# Autodesk Inventor assembly: Cube
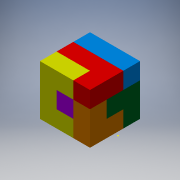
[picture p0: Inventor's stored thumbnail of the model, 180x180]
Saved by Autodesk Inventor 2017 (Build 210142000, 142)
## iProperties
Created: 2016-11-02
Part Number: Cube
Document SubType Name: Assembly
Designer: rbibb
Author: rbibb
## Documents named in this file (7)
- A:\rbibb\School\9th\Enginering\Cube.iam
- A:\rbibb\School\9th\Enginering\Blue part.ipt
- A:\rbibb\School\9th\Enginering\Green part.ipt
- A:\rbibb\School\9th\Enginering\Orange part.ipt
- A:\rbibb\School\9th\Enginering\Purple part.ipt
- A:\rbibb\School\9th\Enginering\Red part.ipt
- A:\rbibb\School\9th\Enginering\Yellow part.ipt
## Components (6 placed, 6 different names)
1. Blue part:1 — Mate:10, Flush:4, Flush:5
2. Green part:1 — Mate:7, Mate:8, Mate:9
3. Orange part:1 — Mate:5, Mate:6, Flush:3, Mate:9
4. Purple part:1 — Mate:3, Mate:4, Flush:2, Mate:5, Flush:3, Mate:8
5. Red part:1 — Mate:1, Mate:2, Flush:1, Mate:6, Mate:7, Mate:10, Flush:4, Flush:5
6. Yellow part:1 — Mate:1, Mate:2, Flush:1, Mate:3, Mate:4, Flush:2
## Relationships (15: Mate 10, Flush 5)
- Mate:1: Red part:1 ↔ Yellow part:1
- Mate:2: Red part:1 ↔ Yellow part:1
- Flush:1: Red part:1 ↔ Yellow part:1
- Mate:3: Purple part:1 ↔ Yellow part:1
- Mate:4: Purple part:1 ↔ Yellow part:1
- Flush:2: Purple part:1 ↔ Yellow part:1
- Mate:5: Orange part:1 ↔ Purple part:1
- Mate:6: Orange part:1 ↔ Red part:1
- Flush:3: Orange part:1 ↔ Purple part:1
- Mate:7: Green part:1 ↔ Red part:1
- Mate:8: Green part:1 ↔ Purple part:1
- Mate:9: Green part:1 ↔ Orange part:1
- Mate:10: Blue part:1 ↔ Red part:1
- Flush:4: Blue part:1 ↔ Red part:1
- Flush:5: Blue part:1 ↔ Red part:1
